# Autodesk Inventor assembly: outer
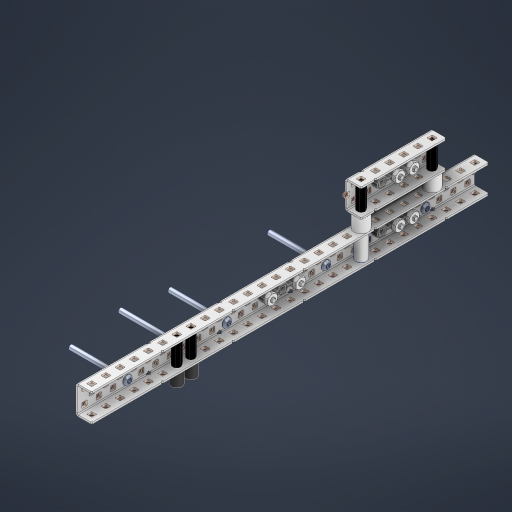
[picture p0: Inventor's stored thumbnail of the model, 512x512]
Saved by Autodesk Inventor 2024 (Build 280153000, 153)
## iProperties
Created: 2023-10-18
Part Number: outer
Document SubType Name: Assembly
Designer: avere
Author: avere
## Documents named in this file (14)
- D:\vex_robotics\hardware\cad\goated_v0.1\chassis\drivebay\outer.iam
- D:\vex_robotics\hardware\cad\VEX-CAD-Inventor-1.41\Structure\C Channel\Aluminum 1x2x1\Alu C 1x2x1x28.ipt
- D:\vex_robotics\hardware\cad\VEX-CAD-Inventor-1.41\Structure\C Channel\Aluminum 1x2x1\Alu C 1x2x1x6.ipt
- D:\vex_robotics\hardware\cad\VEX-CAD-Inventor-1.41\lightweight_offset_bearing.iam
- D:\vex_robotics\hardware\cad\hardware\.375 OD Aluminum Spacer 0.875.ipt
- D:\vex_robotics\hardware\cad\VEX-CAD-Inventor-1.41\Structure\Standoff\Standoff .875.ipt
- C:\Users\avere\Documents\rbp_cad\VEX-CAD-Inventor-1.41\Structure\Standoff.ipt
- D:\vex_robotics\hardware\cad\VEX-CAD-Inventor-1.41\lightweight_bearing.iam
- D:\vex_robotics\hardware\cad\VEX-CAD-Inventor-1.41\Motion\Spacers\Spacer Nylon .375 OD\NSpacer .375 OD x .500.ipt
- C:\Users\avere\Documents\rbp_cad\VEX-CAD-Inventor-1.41\Motion\Spacers\Spacer Nylon .375 OD.ipt
- D:\vex_robotics\hardware\cad\VEX-CAD-Inventor-1.41\Structure\Hardware\Screw Shoulder Robosource\SScrew Shoulder Smooth 2.000 x .04.ipt
- C:\Users\avere\Documents\rbp_cad\VEX-CAD-Inventor-1.41\Structure\Hardware\Screw Shoulder Robosource.ipt
- D:\vex_robotics\hardware\cad\VEX-CAD-Inventor-1.41\Motion\Spacers\Spacer Nylon .500 OD\NSpacer White .500 OD x .500.ipt
- D:\vex_robotics\hardware\cad\VEX-CAD-Inventor-1.41\Motion\Spacers\Spacer Nylon .500 OD.ipt
## Components (19 placed, 9 different names)
1. Alu C 1x2x1x28:1 — Insert:1, Mate:1, Insert:3, Insert:7, Mate:3, Insert:8, Mate:4, Insert:9, Insert:10, Insert:11, Insert:12, Insert:13, Insert:14, Insert:15, Insert:17, Insert:18, Insert:19, Insert:20
2. Alu C 1x2x1x6:1 — Insert:1, Mate:1, Insert:2, Mate:2, Insert:5, Insert:6
3. lightweight_offset_bearing:1 [sub-assembly] — Insert:2, Mate:2
4. .375 OD Aluminum Spacer 0.875:1 — Insert:3
5. Standoff .875:1 — Insert:5
6. Standoff .875:2 — Insert:6
7. lightweight_offset_bearing:2 [sub-assembly] — Insert:7, Mate:3
8. lightweight_bearing:1 [sub-assembly] — Insert:8, Mate:4
9. NSpacer .375 OD x .500:1 — Insert:9
10. NSpacer .375 OD x .500:2 — Insert:10
11. Standoff .875:3 — Insert:11
12. Standoff .875:4 — Insert:12
13. SScrew Shoulder Smooth 2.000 x .04:1 — Insert:13
14. SScrew Shoulder Smooth 2.000 x .04:2 — Insert:14
15. SScrew Shoulder Smooth 2.000 x .04:3 — Insert:15
16. SScrew Shoulder Smooth 2.000 x .04:4 — Insert:18
17. SScrew Shoulder Smooth 2.000 x .04:5 — Insert:17
18. NSpacer White .500 OD x .500:1 — Insert:19
19. NSpacer White .500 OD x .500:2 — Insert:20
## Relationships (22: Insert 18, Mate 4)
- Insert:1 (12.7 mm): Alu C 1x2x1x28:1 ↔ Alu C 1x2x1x6:1
- Mate:1: Alu C 1x2x1x28:1 ↔ Alu C 1x2x1x6:1
- Insert:2: Alu C 1x2x1x6:1 ↔ lightweight_offset_bearing:1
- Mate:2: Alu C 1x2x1x6:1 ↔ lightweight_offset_bearing:1
- Insert:3: Alu C 1x2x1x28:1 ↔ .375 OD Aluminum Spacer 0.875:1
- Insert:5: Alu C 1x2x1x6:1 ↔ Standoff .875:1
- Insert:6: Alu C 1x2x1x6:1 ↔ Standoff .875:2
- Insert:7: Alu C 1x2x1x28:1 ↔ lightweight_offset_bearing:2
- Mate:3: Alu C 1x2x1x28:1 ↔ lightweight_offset_bearing:2
- Insert:8: Alu C 1x2x1x28:1 ↔ lightweight_bearing:1
- Mate:4: Alu C 1x2x1x28:1 ↔ lightweight_bearing:1
- Insert:9: Alu C 1x2x1x28:1 ↔ NSpacer .375 OD x .500:1
- Insert:10: Alu C 1x2x1x28:1 ↔ NSpacer .375 OD x .500:2
- Insert:11: Alu C 1x2x1x28:1 ↔ Standoff .875:3
- Insert:12: Alu C 1x2x1x28:1 ↔ Standoff .875:4
- Insert:13: Alu C 1x2x1x28:1 ↔ SScrew Shoulder Smooth 2.000 x .04:1
- Insert:14: Alu C 1x2x1x28:1 ↔ SScrew Shoulder Smooth 2.000 x .04:2
- Insert:15: Alu C 1x2x1x28:1 ↔ SScrew Shoulder Smooth 2.000 x .04:3
- Insert:17: Alu C 1x2x1x28:1 ↔ SScrew Shoulder Smooth 2.000 x .04:5
- Insert:18: Alu C 1x2x1x28:1 ↔ SScrew Shoulder Smooth 2.000 x .04:4
- Insert:19: Alu C 1x2x1x28:1 ↔ NSpacer White .500 OD x .500:1
- Insert:20: Alu C 1x2x1x28:1 ↔ NSpacer White .500 OD x .500:2
